# Autodesk Inventor assembly: DisplayConcept
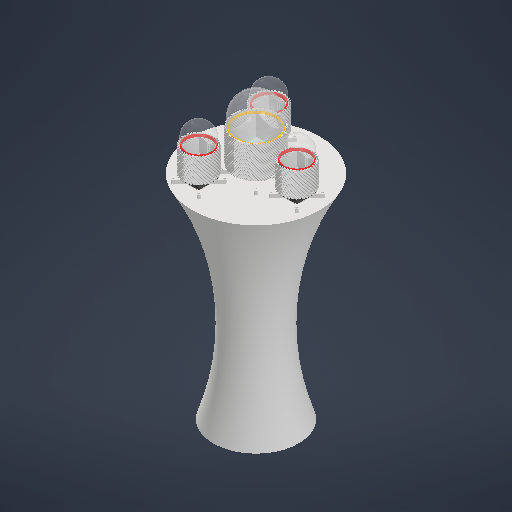
[picture p0: Inventor's stored thumbnail of the model, 512x512]
Saved by Autodesk Inventor 2026 (Build 300175050, 175E)
## iProperties
Created: 2025-06-26
Part Number: DisplayConcept
Document SubType Name: Assembly
Designer: user
Author: user
## Documents named in this file (4)
- C:\Projects\PlasmaTransformer\3D Visual Models\DisplayConcept.iam
- C:\Projects\PlasmaTransformer\3D Visual Models\4xDisplay.ipt
- C:\Projects\PlasmaTransformer\3D Print and CNC\Corrugated-FanShroud-20cm.ipt
- C:\Projects\PlasmaTransformer\3D Print and CNC\Corrugated-FanShroud-13cm.ipt
## Components (5 placed, 3 different names)
1. 4xDisplay:1 — Flush:1, Flush:2, Flush:3, Mate:1, Mate:2, Mate:3, Mate:4, Mate:5, Mate:6, Mate:7
2. Corrugated-FanShroud-20cm:1 — Mate:5
3. Corrugated-FanShroud-13cm:1 — Mate:7
4. Corrugated-FanShroud-13cm:2
5. Corrugated-FanShroud-13cm:3
## Component patterns: (3 elements, first: Corrugated-FanShroud-13cm:1)
## Relationships (10: Mate 7, Flush 3)
- Flush:1: 4xDisplay:1
- Flush:2: 4xDisplay:1
- Flush:3: 4xDisplay:1
- Mate:1: 4xDisplay:1
- Mate:2: 4xDisplay:1
- Mate:3: 4xDisplay:1
- Mate:4: 4xDisplay:1
- Mate:5: 4xDisplay:1 ↔ Corrugated-FanShroud-20cm:1
- Mate:6: 4xDisplay:1
- Mate:7: 4xDisplay:1 ↔ Corrugated-FanShroud-13cm:1
